# Autodesk Inventor assembly: WingAssembly
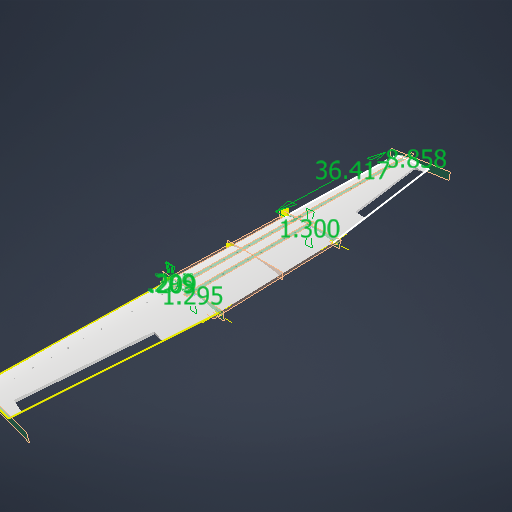
[picture p0: Inventor's stored thumbnail of the model, 512x512]
Saved by Autodesk Inventor 2026 (Build 300175050, 175E)
## iProperties
Created: 2025-06-04
Part Number: WingAssembly
Document SubType Name: Assembly
Designer: Cupri
Author: Cupri
## Documents named in this file (4)
- C:\Users\Delbe\OneDrive\Documents\GitHub\SWIFT-UAV\System_development\Pelican\v0.2\SubAssemblies\WingAssembly\WingAssembly.iam
- C:\Users\Delbe\OneDrive\Documents\GitHub\SWIFT-UAV\System_development\Pelican\v0.2\Parts\MiddleWing.ipt
- C:\Users\Delbe\OneDrive\Documents\GitHub\SWIFT-UAV\System_development\Pelican\v0.2\Parts\OuterWingRight.ipt
- C:\Users\Delbe\OneDrive\Documents\GitHub\SWIFT-UAV\System_development\Pelican\v0.2\Parts\OuterWingLeft.ipt
## Components (3 placed, 3 different names)
1. MiddleWing:1 — Mate:1, Mate:2
2. OuterWingRight:1 — Mate:1, Mate:2
3. OuterWingLeft:1
## Relationships (2: Mate 2)
- Mate:1: MiddleWing:1 ↔ OuterWingRight:1
- Mate:2: MiddleWing:1 ↔ OuterWingRight:1
